# Autodesk Inventor assembly: SPOT_FINAL
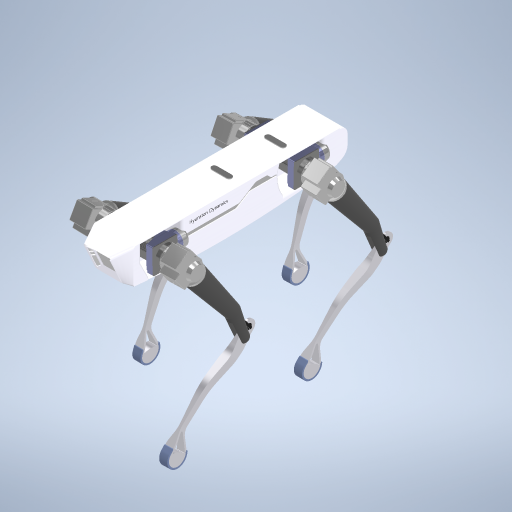
[picture p0: Inventor's stored thumbnail of the model, 512x512]
Saved by Autodesk Inventor 2023 (Build 270158000, 158)
## iProperties
Created: 2022-11-08
Part Number: SPOT_FINAL
Document SubType Name: Assembly
Designer: willy
Author: willy
## Documents named in this file (4)
- C:\Users\willy\Documents\SPOT\SPOT_FINAL.iam
- C:\Users\willy\Documents\SPOT\spot_body.ipt
- C:\Users\willy\Documents\SPOT\RIGHT ARM.iam
- C:\Users\willy\Documents\SPOT\LEFT ARM.iam
## Components (5 placed, 3 different names)
1. spot_body:1 — 삽입:1, 삽입:2, 삽입:3, 삽입:4
2. RIGHT ARM:1 [sub-assembly] — 삽입:1
3. RIGHT ARM:2 [sub-assembly] — 삽입:2
4. LEFT ARM:1 [sub-assembly] — 삽입:3
5. LEFT ARM:2 [sub-assembly] — 삽입:4
## Relationships (4: Insert 4)
- 삽입:1 [Insert]: spot_body:1 ↔ RIGHT ARM:1
- 삽입:2 [Insert]: spot_body:1 ↔ RIGHT ARM:2
- 삽입:3 [Insert]: spot_body:1 ↔ LEFT ARM:1
- 삽입:4 [Insert]: spot_body:1 ↔ LEFT ARM:2
